# Autodesk Inventor assembly: Leg
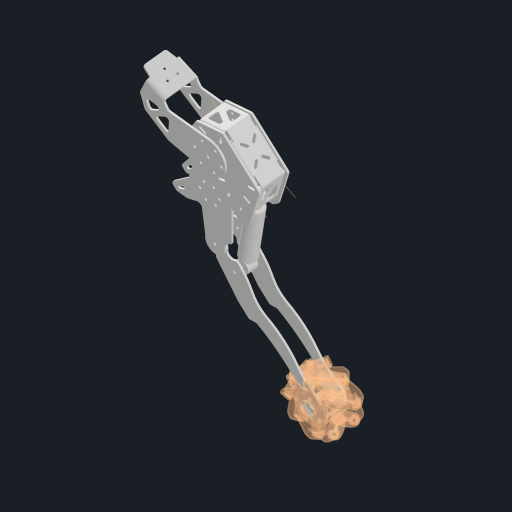
[picture p0: Inventor's stored thumbnail of the model, 512x512]
Saved by Autodesk Inventor 2023 (Build 270158000, 158)
## iProperties
Created: 2020-05-17
Part Number: Leg
Document SubType Name: Assembly
Designer: valer
Author: valer
## Documents named in this file (8)
- C:\Users\valer\Desktop\str1ker\cad\Leg.iam
- C:\Users\valer\Desktop\str1ker\cad\Knee.ipt
- C:\Users\valer\Desktop\str1ker\cad\LowerLeg.ipt
- C:\Users\valer\Desktop\str1ker\cad\UpperLeg.ipt
- C:\Users\valer\Desktop\str1ker\cad\Hip.ipt
- C:\Users\valer\Desktop\str1ker\cad\HipCoverTop.ipt
- C:\Users\valer\Desktop\str1ker\cad\external\MecanumWheel\Mecanum Wheel Derived.ipt
- C:\Users\valer\Desktop\str1ker\cad\external\MecanumWheel\LegShock.ipt
## Components (10 placed, 7 different names)
1. Knee:1 — Flush:1, Mate:1, Mate:3, Mate:4, Angle:1, Mate:14
2. LowerLeg:1 — Mate:3, Angle:1, Mate:14, Mate:21, Mate:22, Mate:23
3. UpperLeg:1 — Flush:1, Mate:1, Mate:4, Mate:5, Mate:6, Mate:7, Mate:16, Mate:17, Mate:18, Mate:19, Mate:20
4. Hip:1 — Mate:5, Mate:6, Mate:7, Mate:11, Mate:12, Mate:13
5. Knee:2 — Mate:15
6. LowerLeg:2 — Mate:15
7. UpperLeg:2 — Mate:11, Mate:12, Mate:13
8. HipCoverTop:1 — Mate:16, Mate:17, Mate:18
9. Mecanum Wheel Derived:1 — Mate:22, Mate:23
10. LegShock:1 — Mate:19, Mate:20, Mate:21
## Relationships (26: Mate 22, Flush 2, Angle 2)
- Flush:1 (-5.08 mm): Knee:1 ↔ UpperLeg:1
- Mate:1: Knee:1 ↔ UpperLeg:1
- Mate:3: Knee:1 ↔ LowerLeg:1
- Mate:4: Knee:1 ↔ UpperLeg:1
- Mate:5: UpperLeg:1 ↔ Hip:1
- Mate:6: UpperLeg:1 ↔ Hip:1
- Mate:7: UpperLeg:1 ↔ Hip:1
- Angle:1 (-40 deg): Knee:1 ↔ LowerLeg:1
- [Flush] (5.08 mm): Knee:2 ↔ UpperLeg:2
- [Mate]: Knee:2 ↔ UpperLeg:2
- [Mate]: Knee:2 ↔ LowerLeg:2
- [Mate]: Knee:2 ↔ UpperLeg:2
- [Angle] (-40 deg): Knee:2 ↔ LowerLeg:2
- Mate:11: Hip:1 ↔ UpperLeg:2
- Mate:12: Hip:1 ↔ UpperLeg:2
- Mate:13: Hip:1 ↔ UpperLeg:2
- Mate:14: Knee:1 ↔ LowerLeg:1
- Mate:15: Knee:2 ↔ LowerLeg:2
- Mate:16: UpperLeg:1 ↔ HipCoverTop:1
- Mate:17: UpperLeg:1 ↔ HipCoverTop:1
- Mate:18: UpperLeg:1 ↔ HipCoverTop:1
- Mate:19: UpperLeg:1 ↔ LegShock:1
- Mate:20 (24.13 mm): UpperLeg:1 ↔ LegShock:1
- Mate:21: LowerLeg:1 ↔ LegShock:1
- Mate:22: LowerLeg:1 ↔ Mecanum Wheel Derived:1
- Mate:23 (12.7 mm): LowerLeg:1 ↔ Mecanum Wheel Derived:1
## Named parameters: d10_d9 = -40 deg, d11_d0 = 5.08 mm, d12_d1 = 0 mm, d14_d4 = 0 mm, d15_d5 = 0 mm
